# Autodesk Inventor assembly: Elevator
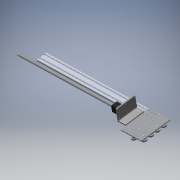
[picture p0: Inventor's stored thumbnail of the model, 180x180]
Saved by Autodesk Inventor 2017 (Build 210142000, 142)
## iProperties
Created: 2016-12-12
Part Number: Elevator
Document SubType Name: Assembly
Designer: umr
Mass: 4376.08 g
Surface Area: 10170.9 cm^2
Volume: 1553.17 cm^3
Density: 2.81752 g/cm^3
Author: umr
## Documents named in this file (9)
- D:\SeniorProject\Models2\Gantry\GantryDown.iam
- D:\SeniorProject\Models2\Gantry\M5 Screw with Tee Nut.iam
- D:\SeniorProject\Models2\Gantry\L_Fixer.ipt
- D:\SeniorProject\Models2\Gantry\ScrewDriver.ipt
- D:\SeniorProject\Models2\Gantry\Motor.ipt
- D:\SeniorProject\Models2\Gantry\GantryPlate_v3.ipt
- D:\SeniorProject\Models2\30x60Sigma.ipt
- D:\SeniorProject\Models2\WheelAssembly\OurWheelAssembly.iam
- D:\SeniorProject\Models2\WheelAssembly\OurWheelAssemblyBig.iam
## Components (21 placed, 8 different names)
1. ScrewDriver:1 — Mate:72, Mate:190
2. Motor:1 — Mate:72, Mate:190, Flush:2, Mate:197, Flush:3
3. GantryPlate_v3:1 — Mate:175, Mate:176, Mate:177, Mate:178, Mate:191, Mate:192, Mate:193, Mate:194, Mate:195, Mate:196
4. 30x60Sigma:1 — Mate:157, Mate:158, Mate:159, Mate:160, Mate:165, Mate:166, Mate:170, Mate:171, Mate:181, Mate:182, Mate:183, Mate:184, Mate:186, Mate:193
5. M5 Screw with Tee Nut:24 [sub-assembly] — Mate:157, Mate:171, Mate:195
6. M5 Screw with Tee Nut:25 [sub-assembly] — Mate:158, Mate:170, Mate:192
7. M5 Screw with Tee Nut:26 [sub-assembly] — Mate:159, Mate:165, Mate:191
8. M5 Screw with Tee Nut:27 [sub-assembly] — Mate:160, Mate:166, Mate:194
9. M5 Screw with Tee Nut:28 [sub-assembly] — Mate:196
10. L_Fixer:1 — Mate:185, Mate:186, Mate:187, Flush:2, Mate:197, Flush:3
11. M5 Screw with Tee Nut:29 [sub-assembly] — Mate:181, Mate:184, Mate:187
12. M5 Screw with Tee Nut:30 [sub-assembly] — Mate:182, Mate:183, Mate:185
13. OurWheelAssembly:1 [sub-assembly] — Mate:175, Mate:176
14. OurWheelAssembly:2 [sub-assembly]
15. OurWheelAssembly:3 [sub-assembly]
16. OurWheelAssembly:4 [sub-assembly]
17. OurWheelAssembly:5 [sub-assembly]
18. OurWheelAssemblyBig:1 [sub-assembly] — Mate:177, Mate:178
19. OurWheelAssemblyBig:2 [sub-assembly]
20. OurWheelAssemblyBig:3 [sub-assembly]
21. OurWheelAssemblyBig:4 [sub-assembly]
## Component patterns: (5 elements, first: OurWheelAssembly:1), (4 elements, first: OurWheelAssemblyBig:1)
## Relationships (30: Mate 28, Flush 2)
- Mate:72: ScrewDriver:1 ↔ Motor:1
- Mate:157: 30x60Sigma:1 ↔ M5 Screw with Tee Nut:24
- Mate:158: 30x60Sigma:1 ↔ M5 Screw with Tee Nut:25
- Mate:159: 30x60Sigma:1 ↔ M5 Screw with Tee Nut:26
- Mate:160: 30x60Sigma:1 ↔ M5 Screw with Tee Nut:27
- Mate:165 (3 mm): 30x60Sigma:1 ↔ M5 Screw with Tee Nut:26
- Mate:166 (3 mm): 30x60Sigma:1 ↔ M5 Screw with Tee Nut:27
- Mate:170 (3 mm): 30x60Sigma:1 ↔ M5 Screw with Tee Nut:25
- Mate:171 (3 mm): 30x60Sigma:1 ↔ M5 Screw with Tee Nut:24
- Mate:175: GantryPlate_v3:1 ↔ OurWheelAssembly:1
- Mate:176: GantryPlate_v3:1 ↔ OurWheelAssembly:1
- Mate:177: GantryPlate_v3:1 ↔ OurWheelAssemblyBig:1
- Mate:178: GantryPlate_v3:1 ↔ OurWheelAssemblyBig:1
- Mate:181 (3 mm): 30x60Sigma:1 ↔ M5 Screw with Tee Nut:29
- Mate:182 (3 mm): 30x60Sigma:1 ↔ M5 Screw with Tee Nut:30
- Mate:183 (2 mm): 30x60Sigma:1 ↔ M5 Screw with Tee Nut:30
- Mate:184 (3 mm): 30x60Sigma:1 ↔ M5 Screw with Tee Nut:29
- Mate:185: L_Fixer:1 ↔ M5 Screw with Tee Nut:30
- Mate:186: 30x60Sigma:1 ↔ L_Fixer:1
- Mate:187: L_Fixer:1 ↔ M5 Screw with Tee Nut:29
- Mate:190: ScrewDriver:1 ↔ Motor:1
- Flush:2 (10 mm): Motor:1 ↔ L_Fixer:1
- Mate:191: GantryPlate_v3:1 ↔ M5 Screw with Tee Nut:26
- Mate:192: GantryPlate_v3:1 ↔ M5 Screw with Tee Nut:25
- Mate:193: GantryPlate_v3:1 ↔ 30x60Sigma:1
- Mate:194: GantryPlate_v3:1 ↔ M5 Screw with Tee Nut:27
- Mate:195: GantryPlate_v3:1 ↔ M5 Screw with Tee Nut:24
- Mate:196: GantryPlate_v3:1 ↔ M5 Screw with Tee Nut:28
- Mate:197: Motor:1 ↔ L_Fixer:1
- Flush:3 (10 mm): Motor:1 ↔ L_Fixer:1
